# Autodesk Inventor assembly: Hip
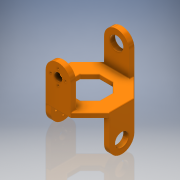
[picture p0: Inventor's stored thumbnail of the model, 180x180]
Saved by Autodesk Inventor 2017 (Build 210142000, 142)
## iProperties
Created: 2017-01-26
Part Number: Hip
Document SubType Name: Assembly
Designer: Alexander Miller
Author: Alexander Miller
## Documents named in this file (2)
- D:\Daten\Documents\Git\Hexapod\3DParts\HexPi_v2\Hip.iam
- D:\Daten\Documents\Git\Hexapod\3DParts\HexPi_v2\Hipjoint.ipt
## Components (2 placed, 1 different names)
1. Hipjoint:1 — Rigid:1
2. Hipjoint:2 — Rigid:1
## Relationships (1: WeldJoint 1)
- Rigid:1 [WeldJoint]: Hipjoint:1 ↔ Hipjoint:2
